# Autodesk Inventor assembly: sorting support
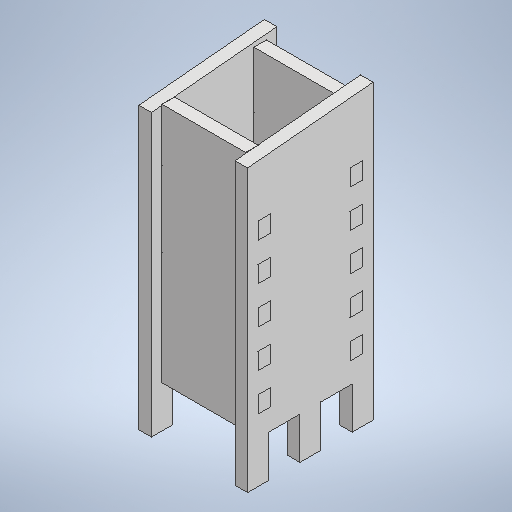
[picture p0: Inventor's stored thumbnail of the model, 512x512]
Saved by Autodesk Inventor 2025.3 (Build 293356000, 356)
## iProperties
Created: 2026-04-27
Part Number: sorting support
Document SubType Name: Assembly
Designer: kamal
Author: kamal
## Documents named in this file (4)
- C:\Users\kamal\OneDrive\Desktop\Personal\semester 4\Basics of Mechatronics\Full Assembly\sorting support.iam
- C:\Users\kamal\OneDrive\Desktop\Personal\semester 4\Basics of Mechatronics\Full Assembly\sort support wall 1.ipt
- C:\Users\kamal\OneDrive\Desktop\Personal\semester 4\Basics of Mechatronics\Full Assembly\sort support wall 2.ipt
- C:\Users\kamal\OneDrive\Desktop\Personal\semester 4\Basics of Mechatronics\Full Assembly\sort support wall 3.ipt
## Components (4 placed, 3 different names)
1. sort support wall 1:1 — Mate:1, Mate:2, Mate:3, Mate:4
2. sort support wall 1:2 — Mate:5, Mate:6
3. sort support wall 2:1 — Mate:3, Mate:4, Mate:5, Mate:6
4. sort support wall 3:1 — Mate:1, Mate:2
## Relationships (6: Mate 6)
- Mate:1: sort support wall 1:1 ↔ sort support wall 3:1
- Mate:2: sort support wall 1:1 ↔ sort support wall 3:1
- Mate:3: sort support wall 1:1 ↔ sort support wall 2:1
- Mate:4: sort support wall 1:1 ↔ sort support wall 2:1
- Mate:5: sort support wall 1:2 ↔ sort support wall 2:1
- Mate:6: sort support wall 1:2 ↔ sort support wall 2:1
